# Autodesk Inventor assembly: Assembly_Cube_BaslerCam_acA1920_25gm_v3
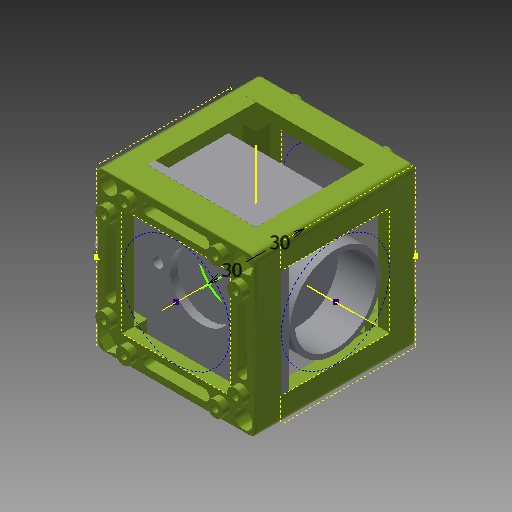
[picture p0: Inventor's stored thumbnail of the model, 512x512]
Saved by Autodesk Inventor 2019 (Build 230136000, 136)
## iProperties
Created: 2019-07-23
Part Number: Assembly_Cube_BaslerCam_acA1920_25gm_v3
Document SubType Name: Assembly
Designer: marsikovabarbora
Author: marsikovabarbora
## Documents named in this file (4)
- C:\Users\marsikovabarbora\Dropbox\UC2\02_CAD\INVENTOR\uc2_v3\Assembly_Cube_BaslerCam_acA1920_25gm_v3.iam
- C:\Users\marsikovabarbora\Dropbox\UC2\02_CAD\INVENTOR\uc2_v3\00_Basler_acA1920_25gm.ipt
- C:\Users\marsikovabarbora\Dropbox\UC2\02_CAD\INVENTOR\uc2_v3\20_Cube_insert_Basler_acA1920_25gm_v3.ipt
- C:\Users\marsikovabarbora\Dropbox\UC2\02_CAD\INVENTOR\uc2_v3\Assembly_Cube_empty_IM_v3.iam
## Components (3 placed, 3 different names)
1. Assembly_Cube_empty_IM_v3:1 [sub-assembly] — Passend:6, Passend:7, Winkel:1, Passend:8
2. 00_Basler_acA1920_25gm:1 — Passend:8, Passend:9
3. 20_Cube_insert_Basler_acA1920_25gm_v3:1 — Passend:6, Passend:7, Winkel:1, Passend:9
## Relationships (8: Mate 7, Angle 1)
- [Mate]: Assembly_Cube_empty_IM_v3:1
- [Mate]: Assembly_Cube_empty_IM_v3:1
- [Mate]: Assembly_Cube_empty_IM_v3:1
- Passend:6 [Mate]: Assembly_Cube_empty_IM_v3:1 ↔ 20_Cube_insert_Basler_acA1920_25gm_v3:1
- Passend:7 [Mate]: Assembly_Cube_empty_IM_v3:1 ↔ 20_Cube_insert_Basler_acA1920_25gm_v3:1
- Winkel:1 [Angle] (0 deg): Assembly_Cube_empty_IM_v3:1 ↔ 20_Cube_insert_Basler_acA1920_25gm_v3:1
- Passend:8 [Mate]: Assembly_Cube_empty_IM_v3:1 ↔ 00_Basler_acA1920_25gm:1
- Passend:9 [Mate]: 00_Basler_acA1920_25gm:1 ↔ 20_Cube_insert_Basler_acA1920_25gm_v3:1
